# Autodesk Inventor assembly: Assembly1
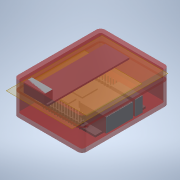
[picture p0: Inventor's stored thumbnail of the model, 180x180]
Saved by Autodesk Inventor 2020 (Build 240168000, 168)
## iProperties
Created: 2019-03-25
Part Number: Assembly1
Document SubType Name: Assembly
Designer: erwin
Author: erwin
## Documents named in this file (3)
- D:\GitHub\ElCheapoAIS-nmea\case\OrangeR1\source\full_assembly.iam
- D:\GitHub\ElCheapoAIS-nmea\case\OrangeR1\source\Imported Components\orangepizero\orangepizero.ipt
- D:\GitHub\ElCheapoAIS-nmea\case\OrangeR1\source\bottom.ipt
## Components (2 placed, 2 different names)
1. orangepizero:1 — Flush:2
2. bottom:1 — Flush:2
## Relationships (1: Flush 1)
- Flush:2 (2 mm): orangepizero:1 ↔ bottom:1
